# Autodesk Inventor assembly: sestaveny dum
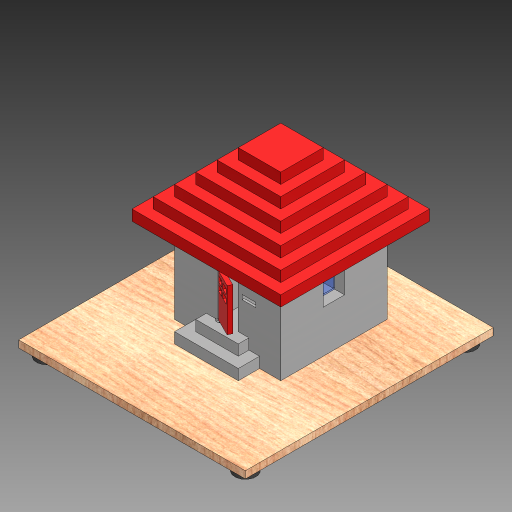
[picture p0: Inventor's stored thumbnail of the model, 512x512]
Saved by Autodesk Inventor 2023 (Build 270158000, 158)
## iProperties
Created: 2022-10-19
Part Number: sestaveny dum
Document SubType Name: Assembly
Designer: zak
Mass: 6542.84 g
Surface Area: 5805.75 cm^2
Volume: 4799.21 cm^3
Density: 1.36331 g/cm^3
Author: zak
## Documents named in this file (7)
- C:\Users\matej\Documents\GitHub\MinecraftBaracek69\model domu\sestaveny dum.iam
- C:\Users\matej\Documents\GitHub\MinecraftBaracek69\model domu\deska.ipt
- C:\Users\matej\Documents\GitHub\MinecraftBaracek69\model domu\steny.ipt
- C:\Users\matej\Documents\GitHub\MinecraftBaracek69\model domu\strecha.ipt
- C:\Users\matej\Documents\GitHub\MinecraftBaracek69\model domu\sklo.ipt
- C:\Users\matej\Documents\GitHub\MinecraftBaracek69\model domu\pacicka.ipt
- C:\Users\matej\Documents\GitHub\MinecraftBaracek69\model domu\dvere.ipt
## Components (9 placed, 6 different names)
1. deska:1 — Proti sobě:1, Vložit:2, Vložit:3, Proti sobě:9, Vložit:4, Proti sobě:10, Proti sobě:11, Proti sobě:12, Vložit:5, Vložit:6, Vložit:7
2. steny:1 — Proti sobě:1, Vložit:2, Vložit:3, Proti sobě:6, Proti sobě:7, Proti sobě:8, Proti sobě:13, Vložit:8, Vložit:9, Proti sobě:14, Proti sobě:15, Proti sobě:16
3. sklo:1 — Proti sobě:6, Proti sobě:7, Proti sobě:8
4. pacicka:1 — Proti sobě:11, Vložit:7
5. pacicka:2 — Proti sobě:12, Vložit:6
6. pacicka:3 — Proti sobě:10, Vložit:5
7. pacicka:4 — Proti sobě:9, Vložit:4
8. dvere:1 — Proti sobě:13, Vložit:8, Vložit:9
9. strecha:1 — Proti sobě:14, Proti sobě:15, Proti sobě:16
## Relationships (20: Mate 12, Insert 8)
- Proti sobě:1 [Mate]: deska:1 ↔ steny:1
- Vložit:2 [Insert]: deska:1 ↔ steny:1
- Vložit:3 [Insert]: deska:1 ↔ steny:1
- Proti sobě:6 [Mate]: steny:1 ↔ sklo:1
- Proti sobě:7 [Mate]: steny:1 ↔ sklo:1
- Proti sobě:8 [Mate]: steny:1 ↔ sklo:1
- Proti sobě:9 [Mate]: deska:1 ↔ pacicka:4
- Vložit:4 [Insert]: deska:1 ↔ pacicka:4
- Proti sobě:10 [Mate]: deska:1 ↔ pacicka:3
- Proti sobě:11 [Mate]: deska:1 ↔ pacicka:1
- Proti sobě:12 [Mate]: deska:1 ↔ pacicka:2
- Vložit:5 [Insert]: deska:1 ↔ pacicka:3
- Vložit:6 [Insert]: deska:1 ↔ pacicka:2
- Vložit:7 [Insert]: deska:1 ↔ pacicka:1
- Proti sobě:13 [Mate]: steny:1 ↔ dvere:1
- Vložit:8 [Insert]: steny:1 ↔ dvere:1
- Vložit:9 [Insert]: steny:1 ↔ dvere:1
- Proti sobě:14 [Mate]: steny:1 ↔ strecha:1
- Proti sobě:15 [Mate]: steny:1 ↔ strecha:1
- Proti sobě:16 [Mate]: steny:1 ↔ strecha:1
